# Autodesk Inventor assembly: camTriggerV02
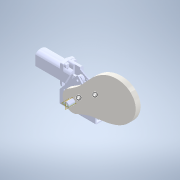
[picture p0: Inventor's stored thumbnail of the model, 180x180]
Saved by Autodesk Inventor 2020.2 (Build 242310000, 310)
## iProperties
Created: 2020-01-12
Part Number: camTriggerV02
Document SubType Name: Assembly
Designer: robst
Author: robst
## Documents named in this file (4)
- C:\git\CAD-Development\robSteele\2020BallTriggerMechanism\camTriggerV02.iam
- C:\git\CAD-Development\robSteele\2020BallTriggerMechanism\am-2235a Snow Blower Motor With Hex Shaft.iam
- C:\git\CAD-Development\robSteele\2020BallTriggerMechanism\am-2373 Snow Blower Motor Mount.ipt
- C:\git\CAD-Development\robSteele\2020BallTriggerMechanism\Disc Cam4.ipt
## Components (3 placed, 3 different names)
1. am-2235a Snow Blower Motor With Hex Shaft:1 [sub-assembly] — Insert:1, Insert:2, Mate:1
2. am-2373 Snow Blower Motor Mount:1 — Insert:1, Insert:2, Mate:2
3. Disc Cam:1 — Mate:1, Mate:2
## Relationships (4: Insert 2, Mate 2)
- Insert:1: am-2235a Snow Blower Motor With Hex Shaft:1 ↔ am-2373 Snow Blower Motor Mount:1
- Insert:2: am-2235a Snow Blower Motor With Hex Shaft:1 ↔ am-2373 Snow Blower Motor Mount:1
- Mate:1: am-2235a Snow Blower Motor With Hex Shaft:1 ↔ Disc Cam:1
- Mate:2: am-2373 Snow Blower Motor Mount:1 ↔ Disc Cam:1
